# Autodesk Inventor assembly: Allocator for column chromatography
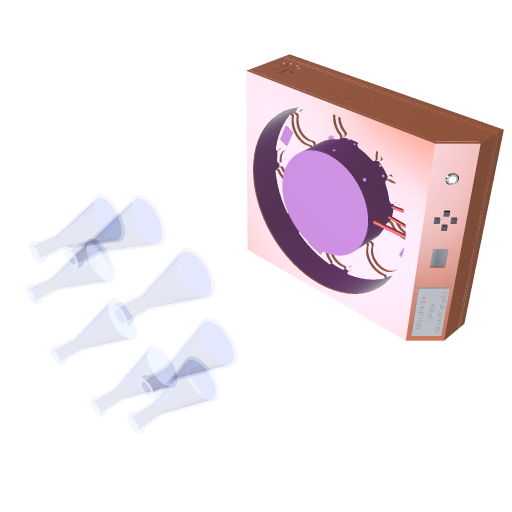
[picture p0: Inventor's stored thumbnail of the model, 512x512]
Saved by Autodesk Inventor 2023 (Build 270158000, 158)
## iProperties
Created: 2023-01-15
Part Number: Allocator for column chromatography
Document SubType Name: Assembly
Designer: Admin
Author: Admin
## Documents named in this file (38)
- C:\Users\aleks\OneDrive\Рабочий стол\Хроматографический сортировщик\Детали\Allocator for column chromatography.iam
- C:\Users\aleks\OneDrive\Рабочий стол\Хроматографический сортировщик\Детали\Барабан.ipt
- C:\Users\aleks\OneDrive\Рабочий стол\Хроматографический сортировщик\Детали\Корпус.ipt
- C:\Users\aleks\OneDrive\Рабочий стол\Хроматографический сортировщик\Детали\Покупные\Болт М5.ipt
- C:\Users\aleks\OneDrive\Рабочий стол\Хроматографический сортировщик\Детали\Покупные\Гайка М5 стопорная.ipt
- C:\Users\aleks\OneDrive\Рабочий стол\Хроматографический сортировщик\Детали\Покупные\Подшипник.ipt
- C:\Users\aleks\OneDrive\Рабочий стол\Хроматографический сортировщик\Детали\Короб подшипника.ipt
- C:\Users\aleks\OneDrive\Рабочий стол\Хроматографический сортировщик\Детали\Покупные\Гайка М3.ipt
- C:\Users\aleks\OneDrive\Рабочий стол\Хроматографический сортировщик\Детали\Покупные\Гайка М4.ipt
- C:\Users\aleks\OneDrive\Рабочий стол\Хроматографический сортировщик\Детали\Покупные\Гайка М6.ipt
- C:\Users\aleks\OneDrive\Рабочий стол\Хроматографический сортировщик\Детали\Покупные\Болт М6.ipt
- C:\Users\aleks\OneDrive\Рабочий стол\Хроматографический сортировщик\Детали\Крепёж оптического датчика.ipt
- C:\Users\aleks\OneDrive\Рабочий стол\Хроматографический сортировщик\Детали\Покупные\Болт М3.ipt
- C:\Users\aleks\OneDrive\Рабочий стол\Хроматографический сортировщик\Детали\Покупные\Болт М4.ipt
- C:\Users\aleks\OneDrive\Рабочий стол\Хроматографический сортировщик\Детали\Покупные\Шаговик\Вал.ipt
- C:\Users\aleks\OneDrive\Рабочий стол\Хроматографический сортировщик\Детали\Покупные\Шаговик\Шаговый мотор.ipt
- C:\Users\aleks\OneDrive\Рабочий стол\Хроматографический сортировщик\Детали\Покупные\Динамик\Динамик.ipt
- C:\Users\aleks\OneDrive\Рабочий стол\Хроматографический сортировщик\Детали\Покупные\Лазер маленький.ipt
- C:\Users\aleks\OneDrive\Рабочий стол\Хроматографический сортировщик\Детали\Покупные\Лазер.ipt
- C:\Users\aleks\OneDrive\Рабочий стол\Хроматографический сортировщик\Детали\Покупные\Оптический датчик.ipt
- C:\Users\aleks\OneDrive\Рабочий стол\Хроматографический сортировщик\Детали\Покупные\Свая.ipt
- C:\Users\aleks\OneDrive\Рабочий стол\Хроматографический сортировщик\Детали\Колесо энкодера.ipt
- C:\Users\aleks\OneDrive\Рабочий стол\Хроматографический сортировщик\Детали\Шевронная маленькая шестерня под мотор.ipt
- C:\Users\aleks\OneDrive\Рабочий стол\Хроматографический сортировщик\Детали\Шевронная планетарная шестерня.ipt
- C:\Users\aleks\OneDrive\Рабочий стол\Хроматографический сортировщик\Детали\Шевронная шестерня для энкодера.ipt
- C:\Users\aleks\OneDrive\Рабочий стол\Хроматографический сортировщик\Детали\Табличка.ipt
- C:\Users\aleks\OneDrive\Рабочий стол\Хроматографический сортировщик\Детали\Покупные\Дисплей.ipt
- C:\Users\aleks\OneDrive\Рабочий стол\Хроматографический сортировщик\Детали\Покупные\Кнопка.ipt
- C:\Users\aleks\OneDrive\Рабочий стол\Хроматографический сортировщик\Детали\Покупные\Кнопки на плате.iam
- C:\Users\aleks\OneDrive\Рабочий стол\Хроматографический сортировщик\Детали\Покупные\Плата главная.ipt
- C:\Users\aleks\OneDrive\Рабочий стол\Хроматографический сортировщик\Детали\Покупные\Разъём питания.ipt
- C:\Users\aleks\OneDrive\Рабочий стол\Хроматографический сортировщик\Детали\Покупные\Болт М2.ipt
- C:\Users\aleks\OneDrive\Рабочий стол\Хроматографический сортировщик\Детали\Покупные\Шаговик\Плата драйвера.ipt
- C:\Users\aleks\OneDrive\Рабочий стол\Хроматографический сортировщик\Детали\Покупные\Болт М3 4мм.ipt
- C:\Users\aleks\OneDrive\Рабочий стол\Хроматографический сортировщик\Детали\Колбы\Модель колба коническая 50мл.ipt
- C:\Users\aleks\OneDrive\Рабочий стол\Хроматографический сортировщик\Детали\Крышка анимации.ipt
- C:\Users\aleks\OneDrive\Рабочий стол\Хроматографический сортировщик\Детали\Покупные\Лазер 2.ipt
- C:\Users\aleks\OneDrive\Рабочий стол\Хроматографический сортировщик\Детали\Покупные\Лазер маленький 2.ipt
## Components (116 placed, 37 different names)
1. Корпус:1 — Совмещение:3, Заподлицо:6, Совмещение:36, Заподлицо:7, Совмещение:37, Угол:2, Заподлицо:8, Заподлицо:9, Совмещение:38, Угол:3, Совмещение:39, Заподлицо:10, Угол:4, Совмещение:40, Совмещение:41, Совмещение:42, Совмещение:43, Совмещение:44, Совмещение:45, Совмещение:46, Совмещение:47, Совмещение:48, Совмещение:49, Заподлицо:11, Заподлицо:12, Заподлицо:13, Заподлицо:14, Заподлицо:15, Заподлицо:16, Заподлицо:17, Заподлицо:18, Заподлицо:19, Заподлицо:20, Заподлицо:21, Заподлицо:22, Угол:5, Угол:6, Угол:7, Угол:8, Угол:9, Угол:10, Угол:11, Угол:12, Угол:13, Угол:14, Совмещение:50, Заподлицо:23, Угол:15, Совмещение:51, Совмещение:52, Совмещение:53, Совмещение:54, Заподлицо:24, Заподлицо:25, Заподлицо:26, Заподлицо:27, Угол:16, Угол:17, Угол:18, Угол:19, Совмещение:55, Совмещение:56, Заподлицо:28, Заподлицо:29, Угол:20, Угол:21, Совмещение:57, Совмещение:58, Заподлицо:30, Заподлицо:31, Угол:22, Угол:23, Совмещение:59, Совмещение:60, Совмещение:61, Совмещение:62, Совмещение:63, Совмещение:64, Совмещение:65, Совмещение:66, Заподлицо:32, Заподлицо:33, Заподлицо:34, Заподлицо:35, Заподлицо:36, Заподлицо:37, Заподлицо:38, Заподлицо:39, Совмещение:69, Совмещение:70, Совмещение:71, Совмещение:72, Совмещение:73, Совмещение:74, Совмещение:75, Совмещение:76, Совмещение:77, Совмещение:78, Совмещение:81, Совмещение:82, Совмещение:83, Совмещение:84, Совмещение:85, Совмещение:86, Угол:24, Угол:25, Заподлицо:40, Заподлицо:41, Совмещение:91, Совмещение:104, Совмещение:105, Совмещение:106, Совмещение:107, Совмещение:108, Совмещение:109, Совмещение:110, Совмещение:111, Совмещение:112, Совмещение:113, Совмещение:114, Совмещение:126, Совмещение:132, Совмещение:133, Совмещение:134, Совмещение:135, Угол:29, Совмещение:136, Совмещение:137, Совмещение:138, Совмещение:139, Совмещение:140, Совмещение:142, Совмещение:143, Совмещение:144, Совмещение:147, Совмещение:148, Совмещение:160, Совмещение:164, Совмещение:169, Совмещение:170, Совмещение:171, Совмещение:172, С поворотом:1, Угол:30, Совмещение:190, Заподлицо:67, Совмещение:191, Совмещение:192, Совмещение:193, Совмещение:194
2. Барабан:1 — Совмещение:3, Совмещение:4, Заподлицо:2, Совмещение:5, Совмещение:6, Совмещение:7, Заподлицо:3, Совмещение:8, Совмещение:9, Заподлицо:4, Совмещение:10, Совмещение:11, Заподлицо:5, Заподлицо:6, Совмещение:179, Совмещение:180, Совмещение:181, Совмещение:182, Совмещение:183, Совмещение:184, Совмещение:185, Совмещение:186, Совмещение:187, Касательность:1, Касательность:2, ЗубчПер:5, С поворотом:1, Угол:30, Совмещение:188, Совмещение:189, ЗубчПер:6
3. Болт М5:1 — Совмещение:19, Совмещение:28
4. Гайка М5 стопорная:1 — Совмещение:23, Совмещение:31
5. Подшипник:1 — Совмещение:15, Совмещение:19, Совмещение:22, Совмещение:25
6. Болт М5:2 — Совмещение:16, Совмещение:20, Совмещение:32
7. Гайка М5 стопорная:2 — Совмещение:20, Совмещение:33
8. Подшипник:2 — Совмещение:12, Совмещение:16, Совмещение:27
9. Болт М5:3 — Совмещение:17, Совмещение:21, Совмещение:34
10. Гайка М5 стопорная:3 — Совмещение:21, Совмещение:35
11. Подшипник:3 — Совмещение:13, Совмещение:17, Совмещение:24
12. Болт М5:4 — Совмещение:18, Совмещение:23, Совмещение:30
13. Гайка М5 стопорная:4 — Совмещение:22, Совмещение:29
14. Подшипник:4 — Совмещение:14, Совмещение:18, Совмещение:26
15. Короб подшипника:1 — Совмещение:8, Совмещение:9, Заподлицо:4, Совмещение:12, Совмещение:27, Совмещение:32, Совмещение:33
16. Короб подшипника:2 — Совмещение:6, Совмещение:7, Заподлицо:3, Совмещение:13, Совмещение:24, Совмещение:34, Совмещение:35
17. Короб подшипника:3 — Совмещение:4, Заподлицо:2, Совмещение:5, Совмещение:15, Совмещение:25, Совмещение:28, Совмещение:29
18. Короб подшипника:4 — Совмещение:10, Совмещение:11, Заподлицо:5, Совмещение:14, Совмещение:26, Совмещение:30, Совмещение:31
19. Подшипник:5 — Совмещение:36, Заподлицо:7, Совмещение:119
20. Гайка М3:1 — Совмещение:41, Заподлицо:13, Угол:6
21. Гайка М3:2 — Совмещение:50, Заподлицо:23, Угол:15
22. Гайка М3:3 — Совмещение:40, Заподлицо:14, Угол:5
23. Гайка М3:4 — Совмещение:43, Заподлицо:22, Угол:8
24. Гайка М3:5 — Совмещение:47, Заподлицо:16, Угол:11
25. Гайка М3:6 — Совмещение:48, Заподлицо:17, Угол:13
26. Гайка М3:7 — Совмещение:37, Угол:2, Заподлицо:8
27. Гайка М3:8 — Заподлицо:9, Совмещение:38, Угол:3, Заподлицо:12
28. Гайка М3:9 — Совмещение:44, Заподлицо:19, Угол:9
29. Гайка М3:11 — Совмещение:49, Заподлицо:18, Угол:14
30. Гайка М3:12 — Совмещение:39, Заподлицо:10, Угол:4, Заподлицо:11
31. Гайка М3:13 — Совмещение:42, Заподлицо:21, Угол:7
32. Гайка М3:14 — Совмещение:45, Заподлицо:20, Угол:10
33. Гайка М3:15 — Совмещение:46, Заподлицо:15, Угол:12
34. Гайка М4:1 — Совмещение:56, Заподлицо:28, Угол:21
35. Гайка М6:1 — Совмещение:53, Заподлицо:26, Угол:17
36. Гайка М4:2 — Совмещение:55, Заподлицо:29, Угол:20
37. Гайка М6:2 — Совмещение:52, Заподлицо:24, Угол:19
38. Гайка М6:3 — Совмещение:51, Заподлицо:25, Угол:18
39. Гайка М6:4 — Совмещение:54, Заподлицо:27, Угол:16
40. Болт М6:1 — Совмещение:61, Заподлицо:34
41. Болт М6:2 — Совмещение:60, Заподлицо:39
42. Гайка М6:5 — Совмещение:57, Заподлицо:31, Угол:22
43. Гайка М6:6 — Совмещение:58, Заподлицо:30, Угол:23
44. Болт М6:3 — Совмещение:62, Заподлицо:37
45. Болт М6:4 — Совмещение:59, Заподлицо:38
46. Болт М6:5 — Совмещение:65, Заподлицо:33
47. Болт М6:6 — Совмещение:64, Заподлицо:35, Совмещение:90
48. Болт М6:7 — Совмещение:66, Заподлицо:32
49. Болт М6:8 — Совмещение:63, Заподлицо:36, Совмещение:89
50. Крепёж оптического датчика:1 — Совмещение:69, Совмещение:87, Совмещение:88, Совмещение:115, Совмещение:116, Совмещение:120, Совмещение:122, Совмещение:123, Угол:26, Угол:27, Совмещение:167, Совмещение:168
51. Болт М3:1 — Совмещение:81, Совмещение:84
52. Болт М3:2 — Совмещение:87, Совмещение:167, Совмещение:171
53. Болт М3:3 — Совмещение:72, Заподлицо:53, Заподлицо:54, Совмещение:152, Совмещение:157
54. Болт М3:4 — Совмещение:78, Заподлицо:43
55. Болт М3:5 — Совмещение:82, Совмещение:83
56. Болт М3:6 — Совмещение:73, Заподлицо:53, Совмещение:153, Совмещение:158
57. Болт М3:7 — Совмещение:76, Заподлицо:44, Заподлицо:45, Совмещение:161
58. Болт М3:8 — Совмещение:70, Совмещение:86
59. Болт М3:9 — Совмещение:75, Заподлицо:52, Заподлицо:54, Совмещение:155
60. Болт М3:10 — Совмещение:74, Заподлицо:52, Совмещение:154, Совмещение:156
61. Болт М3:11 — Совмещение:77, Заподлицо:43, Заподлицо:44, Совмещение:162, Совмещение:163
62. Болт М3:12 — Совмещение:88, Совмещение:168, Совмещение:172
63. Болт М3:13 — Совмещение:71, Совмещение:85
64. Гайка М6:7 — Совмещение:90, Угол:24, Заподлицо:41
65. Гайка М6:8 — Совмещение:89, Угол:25, Заподлицо:40
66. Болт М3:14 — Совмещение:91, Заподлицо:45
67. Болт М4:1 — Совмещение:100, Совмещение:102, Совмещение:169
68. Болт М4:2 — Совмещение:101, Совмещение:103, Совмещение:170
69. Вал:1 — Совмещение:98, Совмещение:99, Совмещение:130, Угол:28, Совмещение:131
70. Шаговый мотор:1 — Совмещение:98, Совмещение:99, Совмещение:100, Совмещение:101, Совмещение:102, Совмещение:103, Совмещение:104
71. Динамик:1 — Совмещение:106, Совмещение:108
72. Динамик:2 — Совмещение:105, Совмещение:107
73. Лазер маленький:1 — Совмещение:111, Совмещение:112
74. Лазер маленький:2 — Совмещение:110, Совмещение:113, Касательность:1, Касательность:2
75. Лазер:1 — Совмещение:109, Совмещение:114
76. Оптический датчик:1 — Совмещение:120, Совмещение:121, Совмещение:122, Совмещение:124, Совмещение:125, Совмещение:129
77. Свая:1 — Совмещение:119, Совмещение:126, Совмещение:127, Совмещение:128, ЗубчПер:1
78. Болт М3:15 — Совмещение:116, Совмещение:118, Совмещение:121, Совмещение:125
79. Гайка М3:16 — Совмещение:118, Заподлицо:46, Угол:27
80. Болт М3:16 — Совмещение:115, Совмещение:117, Совмещение:124
81. Гайка М3:17 — Совмещение:117, Заподлицо:46, Совмещение:123, Угол:26
82. Колесо энкодера:1 — Совмещение:127, Совмещение:129, ЗубчПер:3, Совмещение:173, Совмещение:174
83. Шевронная маленькая шестерня под мотор:1 — Совмещение:130, Угол:28, Совмещение:131, Заподлицо:47, Заподлицо:48, ЗубчПер:2, ЗубчПер:4
84. Шевронная шестерня для энкодера:1 — Совмещение:128, Заподлицо:47, ЗубчПер:1, ЗубчПер:2, ЗубчПер:3, Совмещение:175, Совмещение:176
85. Шевронная планетарная шестерня:1 — Совмещение:132, Заподлицо:48, ЗубчПер:4, ЗубчПер:5
86. Табличка:1 — Совмещение:135, Угол:29, Совмещение:136, Совмещение:137
87. Кнопка:1 — Совмещение:138, Совмещение:139
88. Кнопки на плате:1 [sub-assembly] — Совмещение:140, Совмещение:142, Совмещение:143
89. Плата главная:1 — Совмещение:152, Совмещение:153, Совмещение:154, Совмещение:159
90. Разъём питания:1 — Совмещение:133, Совмещение:134
91. Болт М2:1 — Заподлицо:49, Заподлицо:50, Заподлицо:51, Совмещение:145, Совмещение:147, Совмещение:151
92. Болт М2:2 — Заподлицо:49, Совмещение:149
93. Болт М2:3 — Заподлицо:51, Совмещение:146, Совмещение:148
94. Болт М2:4 — Заподлицо:50, Совмещение:150
95. Дисплей:1 — Совмещение:144, Совмещение:145, Совмещение:146, Совмещение:149, Совмещение:150, Совмещение:151
96. Гайка М3:18 — Совмещение:155, Заподлицо:56, Заподлицо:57
97. Гайка М3:19 — Совмещение:156, Заподлицо:55, Заподлицо:57
98. Гайка М3:20 — Совмещение:157, Заподлицо:56
99. Гайка М3:21 — Совмещение:158, Заподлицо:55, Совмещение:159, Совмещение:160
100. Плата драйвера:1 — Совмещение:161, Совмещение:162, Совмещение:163, Совмещение:164
101. Болт М3 4мм:1 — Совмещение:173, Совмещение:174
102. Болт М3 4мм:2 — Совмещение:175, Совмещение:176
103. Подшипник:6
104. Подшипник:7
105. Модель колба коническая 50мл:2 — Совмещение:180, Заподлицо:61, Заподлицо:62
106. Модель колба коническая 50мл:3 — Совмещение:181, Заподлицо:66
107. Модель колба коническая 50мл:4 — Совмещение:182, Заподлицо:60, Заподлицо:61
108. Модель колба коническая 50мл:5 — Совмещение:186, Заподлицо:64
109. Модель колба коническая 50мл:6 — Совмещение:183, Заподлицо:60
110. Модель колба коническая 50мл:7 — Совмещение:184, Заподлицо:65
111. Модель колба коническая 50мл:8 — Совмещение:185, Заподлицо:63
112. Модель колба коническая 50мл:9 — Совмещение:179, Заподлицо:62, Заподлицо:63, Заподлицо:64, Заподлицо:65, Заподлицо:66, Совмещение:187
113. Крышка анимации:1 — Совмещение:188, Совмещение:189, ЗубчПер:6
114. Лазер 2:1 — Совмещение:190, Заподлицо:67
115. Лазер маленький 2:1 — Совмещение:191, Совмещение:194
116. Лазер маленький 2:2 — Совмещение:192, Совмещение:193
## Relationships (278: Mate 177, Flush 63, Angle 29, RelateRotation 6, Tangent 2, RevoluteJoint 1)
- Совмещение:3 [Mate]: Корпус:1 ↔ Барабан:1
- Совмещение:4 [Mate] (0.1 mm): Барабан:1 ↔ Короб подшипника:3
- Заподлицо:2 [Flush]: Барабан:1 ↔ Короб подшипника:3
- Совмещение:5 [Mate] (0.1 mm): Барабан:1 ↔ Короб подшипника:3
- Совмещение:6 [Mate] (0.1 mm): Барабан:1 ↔ Короб подшипника:2
- Совмещение:7 [Mate] (0.1 mm): Барабан:1 ↔ Короб подшипника:2
- Заподлицо:3 [Flush]: Барабан:1 ↔ Короб подшипника:2
- Совмещение:8 [Mate] (0.1 mm): Барабан:1 ↔ Короб подшипника:1
- Совмещение:9 [Mate] (0.1 mm): Барабан:1 ↔ Короб подшипника:1
- Заподлицо:4 [Flush]: Барабан:1 ↔ Короб подшипника:1
- Совмещение:10 [Mate] (0.1 mm): Барабан:1 ↔ Короб подшипника:4
- Совмещение:11 [Mate] (0.1 mm): Барабан:1 ↔ Короб подшипника:4
- Заподлицо:5 [Flush]: Барабан:1 ↔ Короб подшипника:4
- Совмещение:12 [Mate]: Подшипник:2 ↔ Короб подшипника:1
- Совмещение:13 [Mate]: Подшипник:3 ↔ Короб подшипника:2
- Совмещение:14 [Mate]: Подшипник:4 ↔ Короб подшипника:4
- Совмещение:15 [Mate]: Подшипник:1 ↔ Короб подшипника:3
- Совмещение:16 [Mate]: Болт М5:2 ↔ Подшипник:2
- Совмещение:17 [Mate]: Болт М5:3 ↔ Подшипник:3
- Совмещение:18 [Mate]: Болт М5:4 ↔ Подшипник:4
- Совмещение:19 [Mate]: Болт М5:1 ↔ Подшипник:1
- Совмещение:20 [Mate]: Болт М5:2 ↔ Гайка М5 стопорная:2
- Совмещение:21 [Mate]: Болт М5:3 ↔ Гайка М5 стопорная:3
- Совмещение:22 [Mate]: Подшипник:1 ↔ Гайка М5 стопорная:4
- Совмещение:23 [Mate]: Гайка М5 стопорная:1 ↔ Болт М5:4
- Совмещение:24 [Mate] (0.5 mm): Подшипник:3 ↔ Короб подшипника:2
- Совмещение:25 [Mate] (0.5 mm): Подшипник:1 ↔ Короб подшипника:3
- Совмещение:26 [Mate] (0.5 mm): Подшипник:4 ↔ Короб подшипника:4
- Совмещение:27 [Mate] (0.5 mm): Подшипник:2 ↔ Короб подшипника:1
- Совмещение:28 [Mate]: Болт М5:1 ↔ Короб подшипника:3
- Совмещение:29 [Mate]: Гайка М5 стопорная:4 ↔ Короб подшипника:3
- Совмещение:30 [Mate]: Болт М5:4 ↔ Короб подшипника:4
- Совмещение:31 [Mate]: Гайка М5 стопорная:1 ↔ Короб подшипника:4
- Совмещение:32 [Mate]: Болт М5:2 ↔ Короб подшипника:1
- Совмещение:33 [Mate]: Гайка М5 стопорная:2 ↔ Короб подшипника:1
- Совмещение:34 [Mate]: Болт М5:3 ↔ Короб подшипника:2
- Совмещение:35 [Mate]: Гайка М5 стопорная:3 ↔ Короб подшипника:2
- Заподлицо:6 [Flush]: Корпус:1 ↔ Барабан:1
- Совмещение:36 [Mate]: Корпус:1 ↔ Подшипник:5
- Заподлицо:7 [Flush]: Корпус:1 ↔ Подшипник:5
- Совмещение:37 [Mate]: Корпус:1 ↔ Гайка М3:7
- Угол:2 [Angle] (0 deg): Корпус:1 ↔ Гайка М3:7
- Заподлицо:8 [Flush]: Корпус:1 ↔ Гайка М3:7
- Заподлицо:9 [Flush]: Корпус:1 ↔ Гайка М3:8
- Совмещение:38 [Mate]: Корпус:1 ↔ Гайка М3:8
- Угол:3 [Angle] (0 deg): Корпус:1 ↔ Гайка М3:8
- Совмещение:39 [Mate]: Корпус:1 ↔ Гайка М3:12
- Заподлицо:10 [Flush]: Корпус:1 ↔ Гайка М3:12
- Угол:4 [Angle] (0 deg): Корпус:1 ↔ Гайка М3:12
- Совмещение:40 [Mate]: Корпус:1 ↔ Гайка М3:3
- Совмещение:41 [Mate]: Корпус:1 ↔ Гайка М3:1
- Совмещение:42 [Mate]: Корпус:1 ↔ Гайка М3:13
- Совмещение:43 [Mate]: Корпус:1 ↔ Гайка М3:4
- Совмещение:44 [Mate]: Корпус:1 ↔ Гайка М3:9
- Совмещение:45 [Mate]: Корпус:1 ↔ Гайка М3:14
- Совмещение:46 [Mate]: Корпус:1 ↔ Гайка М3:15
- Совмещение:47 [Mate]: Корпус:1 ↔ Гайка М3:5
- Совмещение:48 [Mate]: Корпус:1 ↔ Гайка М3:6
- Совмещение:49 [Mate]: Корпус:1 ↔ Гайка М3:11
- Заподлицо:11 [Flush]: Корпус:1 ↔ Гайка М3:12
- Заподлицо:12 [Flush]: Корпус:1 ↔ Гайка М3:8
- Заподлицо:13 [Flush]: Корпус:1 ↔ Гайка М3:1
- Заподлицо:14 [Flush]: Корпус:1 ↔ Гайка М3:3
- Заподлицо:15 [Flush]: Корпус:1 ↔ Гайка М3:15
- Заподлицо:16 [Flush]: Корпус:1 ↔ Гайка М3:5
- Заподлицо:17 [Flush]: Корпус:1 ↔ Гайка М3:6
- Заподлицо:18 [Flush]: Корпус:1 ↔ Гайка М3:11
- Заподлицо:19 [Flush]: Корпус:1 ↔ Гайка М3:9
- Заподлицо:20 [Flush]: Корпус:1 ↔ Гайка М3:14
- Заподлицо:21 [Flush]: Корпус:1 ↔ Гайка М3:13
- Заподлицо:22 [Flush]: Корпус:1 ↔ Гайка М3:4
- Угол:5 [Angle] (0 deg): Корпус:1 ↔ Гайка М3:3
- Угол:6 [Angle] (0 deg): Корпус:1 ↔ Гайка М3:1
- Угол:7 [Angle] (0 deg): Корпус:1 ↔ Гайка М3:13
- Угол:8 [Angle] (0 deg): Корпус:1 ↔ Гайка М3:4
- Угол:9 [Angle] (0 deg): Корпус:1 ↔ Гайка М3:9
- Угол:10 [Angle] (0 deg): Корпус:1 ↔ Гайка М3:14
- Угол:11 [Angle] (0 deg): Корпус:1 ↔ Гайка М3:5
- Угол:12 [Angle] (0 deg): Корпус:1 ↔ Гайка М3:15
- Угол:13 [Angle] (0 deg): Корпус:1 ↔ Гайка М3:6
- Угол:14 [Angle] (0 deg): Корпус:1 ↔ Гайка М3:11
- Совмещение:50 [Mate]: Корпус:1 ↔ Гайка М3:2
- Заподлицо:23 [Flush]: Корпус:1 ↔ Гайка М3:2
- Угол:15 [Angle] (0 deg): Корпус:1 ↔ Гайка М3:2
- Совмещение:51 [Mate]: Корпус:1 ↔ Гайка М6:3
- Совмещение:52 [Mate]: Корпус:1 ↔ Гайка М6:2
- Совмещение:53 [Mate]: Корпус:1 ↔ Гайка М6:1
- Совмещение:54 [Mate]: Корпус:1 ↔ Гайка М6:4
- Заподлицо:24 [Flush]: Корпус:1 ↔ Гайка М6:2
- Заподлицо:25 [Flush]: Корпус:1 ↔ Гайка М6:3
- Заподлицо:26 [Flush]: Корпус:1 ↔ Гайка М6:1
- Заподлицо:27 [Flush]: Корпус:1 ↔ Гайка М6:4
- Угол:16 [Angle] (0 deg): Корпус:1 ↔ Гайка М6:4
- Угол:17 [Angle] (0 deg): Корпус:1 ↔ Гайка М6:1
- Угол:18 [Angle] (0 deg): Корпус:1 ↔ Гайка М6:3
- Угол:19 [Angle] (0 deg): Корпус:1 ↔ Гайка М6:2
- Совмещение:55 [Mate]: Корпус:1 ↔ Гайка М4:2
- Совмещение:56 [Mate]: Корпус:1 ↔ Гайка М4:1
- Заподлицо:28 [Flush]: Корпус:1 ↔ Гайка М4:1
- Заподлицо:29 [Flush]: Корпус:1 ↔ Гайка М4:2
- Угол:20 [Angle] (0 deg): Корпус:1 ↔ Гайка М4:2
- Угол:21 [Angle] (0 deg): Корпус:1 ↔ Гайка М4:1
- Совмещение:57 [Mate]: Корпус:1 ↔ Гайка М6:5
- Совмещение:58 [Mate]: Корпус:1 ↔ Гайка М6:6
- Заподлицо:30 [Flush]: Корпус:1 ↔ Гайка М6:6
- Заподлицо:31 [Flush]: Корпус:1 ↔ Гайка М6:5
- Угол:22 [Angle] (0 deg): Корпус:1 ↔ Гайка М6:5
- Угол:23 [Angle] (0 deg): Корпус:1 ↔ Гайка М6:6
- Совмещение:59 [Mate]: Корпус:1 ↔ Болт М6:4
- Совмещение:60 [Mate]: Корпус:1 ↔ Болт М6:2
- Совмещение:61 [Mate]: Корпус:1 ↔ Болт М6:1
- Совмещение:62 [Mate]: Корпус:1 ↔ Болт М6:3
- Совмещение:63 [Mate]: Корпус:1 ↔ Болт М6:8
- Совмещение:64 [Mate]: Корпус:1 ↔ Болт М6:6
- Совмещение:65 [Mate]: Корпус:1 ↔ Болт М6:5
- Совмещение:66 [Mate]: Корпус:1 ↔ Болт М6:7
- Заподлицо:32 [Flush]: Корпус:1 ↔ Болт М6:7
- Заподлицо:33 [Flush]: Корпус:1 ↔ Болт М6:5
- Заподлицо:34 [Flush]: Корпус:1 ↔ Болт М6:1
- Заподлицо:35 [Flush]: Корпус:1 ↔ Болт М6:6
- Заподлицо:36 [Flush]: Корпус:1 ↔ Болт М6:8
- Заподлицо:37 [Flush]: Корпус:1 ↔ Болт М6:3
- Заподлицо:38 [Flush]: Корпус:1 ↔ Болт М6:4
- Заподлицо:39 [Flush]: Корпус:1 ↔ Болт М6:2
- Совмещение:69 [Mate]: Корпус:1 ↔ Крепёж оптического датчика:1
- Совмещение:70 [Mate]: Корпус:1 ↔ Болт М3:8
- Совмещение:71 [Mate]: Корпус:1 ↔ Болт М3:13
- Совмещение:72 [Mate]: Корпус:1 ↔ Болт М3:3
- Совмещение:73 [Mate]: Корпус:1 ↔ Болт М3:6
- Совмещение:74 [Mate]: Корпус:1 ↔ Болт М3:10
- Совмещение:75 [Mate]: Корпус:1 ↔ Болт М3:9
- Совмещение:76 [Mate]: Корпус:1 ↔ Болт М3:7
- Совмещение:77 [Mate]: Корпус:1 ↔ Болт М3:11
- Совмещение:78 [Mate]: Корпус:1 ↔ Болт М3:4
- Совмещение:81 [Mate]: Корпус:1 ↔ Болт М3:1
- Совмещение:82 [Mate]: Корпус:1 ↔ Болт М3:5
- Совмещение:83 [Mate]: Корпус:1 ↔ Болт М3:5
- Совмещение:84 [Mate]: Корпус:1 ↔ Болт М3:1
- Совмещение:85 [Mate]: Корпус:1 ↔ Болт М3:13
- Совмещение:86 [Mate]: Корпус:1 ↔ Болт М3:8
- Совмещение:87 [Mate]: Крепёж оптического датчика:1 ↔ Болт М3:2
- Совмещение:88 [Mate]: Крепёж оптического датчика:1 ↔ Болт М3:12
- Совмещение:89 [Mate]: Болт М6:8 ↔ Гайка М6:8
- Совмещение:90 [Mate]: Болт М6:6 ↔ Гайка М6:7
- Угол:24 [Angle] (0 deg): Корпус:1 ↔ Гайка М6:7
- Угол:25 [Angle] (0 deg): Корпус:1 ↔ Гайка М6:8
- Заподлицо:40 [Flush]: Корпус:1 ↔ Гайка М6:8
- Заподлицо:41 [Flush]: Корпус:1 ↔ Гайка М6:7
- Совмещение:91 [Mate]: Корпус:1 ↔ Болт М3:14
- Заподлицо:43 [Flush]: Болт М3:4 ↔ Болт М3:11
- Заподлицо:44 [Flush]: Болт М3:7 ↔ Болт М3:11
- Заподлицо:45 [Flush]: Болт М3:7 ↔ Болт М3:14
- Совмещение:98 [Mate]: Вал:1 ↔ Шаговый мотор:1
- Совмещение:99 [Mate]: Вал:1 ↔ Шаговый мотор:1
- Совмещение:100 [Mate]: Болт М4:1 ↔ Шаговый мотор:1
- Совмещение:101 [Mate]: Болт М4:2 ↔ Шаговый мотор:1
- Совмещение:102 [Mate]: Болт М4:1 ↔ Шаговый мотор:1
- Совмещение:103 [Mate]: Болт М4:2 ↔ Шаговый мотор:1
- Совмещение:104 [Mate]: Корпус:1 ↔ Шаговый мотор:1
- Совмещение:105 [Mate]: Корпус:1 ↔ Динамик:2
- Совмещение:106 [Mate]: Корпус:1 ↔ Динамик:1
- Совмещение:107 [Mate]: Корпус:1 ↔ Динамик:2
- Совмещение:108 [Mate]: Корпус:1 ↔ Динамик:1
- Совмещение:109 [Mate]: Корпус:1 ↔ Лазер:1
- Совмещение:110 [Mate]: Корпус:1 ↔ Лазер маленький:2
- Совмещение:111 [Mate]: Корпус:1 ↔ Лазер маленький:1
- Совмещение:112 [Mate]: Корпус:1 ↔ Лазер маленький:1
- Совмещение:113 [Mate]: Корпус:1 ↔ Лазер маленький:2
- Совмещение:114 [Mate]: Корпус:1 ↔ Лазер:1
- Совмещение:115 [Mate]: Крепёж оптического датчика:1 ↔ Болт М3:16
- Совмещение:116 [Mate]: Крепёж оптического датчика:1 ↔ Болт М3:15
- Совмещение:117 [Mate]: Болт М3:16 ↔ Гайка М3:17
- Совмещение:118 [Mate]: Болт М3:15 ↔ Гайка М3:16
- Совмещение:119 [Mate]: Подшипник:5 ↔ Свая:1
- Совмещение:120 [Mate]: Крепёж оптического датчика:1 ↔ Оптический датчик:1
- Совмещение:121 [Mate]: Оптический датчик:1 ↔ Болт М3:15
- Совмещение:122 [Mate]: Крепёж оптического датчика:1 ↔ Оптический датчик:1
- Заподлицо:46 [Flush]: Гайка М3:16 ↔ Гайка М3:17
- Совмещение:123 [Mate]: Крепёж оптического датчика:1 ↔ Гайка М3:17
- Угол:26 [Angle] (0 deg): Крепёж оптического датчика:1 ↔ Гайка М3:17
- Угол:27 [Angle] (0 deg): Крепёж оптического датчика:1 ↔ Гайка М3:16
- Совмещение:124 [Mate]: Оптический датчик:1 ↔ Болт М3:16
- Совмещение:125 [Mate]: Оптический датчик:1 ↔ Болт М3:15
- Совмещение:126 [Mate]: Корпус:1 ↔ Свая:1
- Совмещение:127 [Mate]: Свая:1 ↔ Колесо энкодера:1
- Совмещение:128 [Mate]: Свая:1 ↔ Шевронная шестерня для энкодера:1
- Совмещение:129 [Mate] (2 mm): Оптический датчик:1 ↔ Колесо энкодера:1
- Совмещение:130 [Mate]: Вал:1 ↔ Шевронная маленькая шестерня под мотор:1
- Угол:28 [Angle] (0 deg): Вал:1 ↔ Шевронная маленькая шестерня под мотор:1
- Совмещение:131 [Mate]: Вал:1 ↔ Шевронная маленькая шестерня под мотор:1
- Заподлицо:47 [Flush]: Шевронная маленькая шестерня под мотор:1 ↔ Шевронная шестерня для энкодера:1
- Совмещение:132 [Mate]: Корпус:1 ↔ Шевронная планетарная шестерня:1
- Заподлицо:48 [Flush]: Шевронная маленькая шестерня под мотор:1 ↔ Шевронная планетарная шестерня:1
- ЗубчПер:1 [RelateRotation] (1 ul): Свая:1 ↔ Шевронная шестерня для энкодера:1
- ЗубчПер:2 [RelateRotation] (1 ul): Шевронная маленькая шестерня под мотор:1 ↔ Шевронная шестерня для энкодера:1
- ЗубчПер:3 [RelateRotation] (1 ul): Колесо энкодера:1 ↔ Шевронная шестерня для энкодера:1
- ЗубчПер:4 [RelateRotation] (0.375 ul): Шевронная маленькая шестерня под мотор:1 ↔ Шевронная планетарная шестерня:1
- Совмещение:133 [Mate]: Корпус:1 ↔ Разъём питания:1
- Совмещение:134 [Mate]: Корпус:1 ↔ Разъём питания:1
- Совмещение:135 [Mate]: Корпус:1 ↔ Табличка:1
- Угол:29 [Angle] (0 deg): Корпус:1 ↔ Табличка:1
- Совмещение:136 [Mate] (5.127 mm): Корпус:1 ↔ Табличка:1
- Совмещение:137 [Mate] (10 mm): Корпус:1 ↔ Табличка:1
- Совмещение:138 [Mate]: Корпус:1 ↔ Кнопка:1
- Совмещение:139 [Mate]: Корпус:1 ↔ Кнопка:1
- Совмещение:140 [Mate]: Корпус:1 ↔ Кнопки на плате:1
- Совмещение:142 [Mate] (0.05 mm): Корпус:1 ↔ Кнопки на плате:1
- Совмещение:143 [Mate] (0.05 mm): Корпус:1 ↔ Кнопки на плате:1
- Заподлицо:49 [Flush]: Болт М2:1 ↔ Болт М2:2
- Заподлицо:50 [Flush]: Болт М2:1 ↔ Болт М2:4
- Заподлицо:51 [Flush]: Болт М2:1 ↔ Болт М2:3
- Совмещение:144 [Mate]: Корпус:1 ↔ Дисплей:1
- Совмещение:145 [Mate]: Болт М2:1 ↔ Дисплей:1
- Совмещение:146 [Mate]: Болт М2:3 ↔ Дисплей:1
- Совмещение:147 [Mate]: Корпус:1 ↔ Болт М2:1
- Совмещение:148 [Mate]: Корпус:1 ↔ Болт М2:3
- Совмещение:149 [Mate]: Болт М2:2 ↔ Дисплей:1
- Совмещение:150 [Mate]: Болт М2:4 ↔ Дисплей:1
- Совмещение:151 [Mate]: Болт М2:1 ↔ Дисплей:1
- Заподлицо:52 [Flush]: Болт М3:9 ↔ Болт М3:10
- Заподлицо:53 [Flush]: Болт М3:3 ↔ Болт М3:6
- Заподлицо:54 [Flush]: Болт М3:3 ↔ Болт М3:9
- Совмещение:152 [Mate]: Болт М3:3 ↔ Плата главная:1
- Совмещение:153 [Mate]: Болт М3:6 ↔ Плата главная:1
- Совмещение:154 [Mate]: Болт М3:10 ↔ Плата главная:1
- Совмещение:155 [Mate]: Болт М3:9 ↔ Гайка М3:18
- Совмещение:156 [Mate]: Болт М3:10 ↔ Гайка М3:19
- Совмещение:157 [Mate]: Болт М3:3 ↔ Гайка М3:20
- Совмещение:158 [Mate]: Болт М3:6 ↔ Гайка М3:21
- Заподлицо:55 [Flush]: Гайка М3:19 ↔ Гайка М3:21
- Заподлицо:56 [Flush]: Гайка М3:18 ↔ Гайка М3:20
- Заподлицо:57 [Flush]: Гайка М3:18 ↔ Гайка М3:19
- Совмещение:159 [Mate]: Плата главная:1 ↔ Гайка М3:21
- Совмещение:160 [Mate]: Корпус:1 ↔ Гайка М3:21
- Совмещение:161 [Mate]: Болт М3:7 ↔ Плата драйвера:1
- Совмещение:162 [Mate]: Болт М3:11 ↔ Плата драйвера:1
- Совмещение:163 [Mate]: Болт М3:11 ↔ Плата драйвера:1
- Совмещение:164 [Mate]: Корпус:1 ↔ Плата драйвера:1
- Совмещение:167 [Mate]: Крепёж оптического датчика:1 ↔ Болт М3:2
- Совмещение:168 [Mate]: Крепёж оптического датчика:1 ↔ Болт М3:12
- Совмещение:169 [Mate]: Корпус:1 ↔ Болт М4:1
- Совмещение:170 [Mate]: Корпус:1 ↔ Болт М4:2
- Совмещение:171 [Mate]: Корпус:1 ↔ Болт М3:2
- Совмещение:172 [Mate]: Корпус:1 ↔ Болт М3:12
- Совмещение:173 [Mate]: Колесо энкодера:1 ↔ Болт М3 4мм:1
- Совмещение:174 [Mate] (2.5 mm): Колесо энкодера:1 ↔ Болт М3 4мм:1
- Совмещение:175 [Mate]: Шевронная шестерня для энкодера:1 ↔ Болт М3 4мм:2
- Совмещение:176 [Mate] (2.5 mm): Шевронная шестерня для энкодера:1 ↔ Болт М3 4мм:2
- Совмещение:179 [Mate]: Барабан:1 ↔ Модель колба коническая 50мл:9
- Совмещение:180 [Mate]: Барабан:1 ↔ Модель колба коническая 50мл:2
- Совмещение:181 [Mate]: Барабан:1 ↔ Модель колба коническая 50мл:3
- Совмещение:182 [Mate]: Барабан:1 ↔ Модель колба коническая 50мл:4
- Совмещение:183 [Mate]: Барабан:1 ↔ Модель колба коническая 50мл:6
- Совмещение:184 [Mate]: Барабан:1 ↔ Модель колба коническая 50мл:7
- Совмещение:185 [Mate]: Барабан:1 ↔ Модель колба коническая 50мл:8
- Совмещение:186 [Mate]: Барабан:1 ↔ Модель колба коническая 50мл:5
- Заподлицо:60 [Flush]: Модель колба коническая 50мл:4 ↔ Модель колба коническая 50мл:6
- Заподлицо:61 [Flush]: Модель колба коническая 50мл:2 ↔ Модель колба коническая 50мл:4
- Заподлицо:62 [Flush]: Модель колба коническая 50мл:2 ↔ Модель колба коническая 50мл:9
- Заподлицо:63 [Flush]: Модель колба коническая 50мл:8 ↔ Модель колба коническая 50мл:9
- Заподлицо:64 [Flush]: Модель колба коническая 50мл:5 ↔ Модель колба коническая 50мл:9
- Заподлицо:65 [Flush]: Модель колба коническая 50мл:7 ↔ Модель колба коническая 50мл:9
- Заподлицо:66 [Flush]: Модель колба коническая 50мл:3 ↔ Модель колба коническая 50мл:9
- Совмещение:187 [Mate] (300 mm): Барабан:1 ↔ Модель колба коническая 50мл:9
- Касательность:1 [Tangent]: Барабан:1 ↔ Лазер маленький:2
- Касательность:2 [Tangent]: Барабан:1 ↔ Лазер маленький:2
- ЗубчПер:5 [RelateRotation] (1 ul): Барабан:1 ↔ Шевронная планетарная шестерня:1
- С поворотом:1 [RevoluteJoint]: Корпус:1 ↔ Барабан:1
- Угол:30 [Angle] (0 deg): Корпус:1 ↔ Барабан:1
- Совмещение:188 [Mate]: Барабан:1 ↔ Крышка анимации:1
- Совмещение:189 [Mate]: Барабан:1 ↔ Крышка анимации:1
- ЗубчПер:6 [RelateRotation] (1 ul): Барабан:1 ↔ Крышка анимации:1
- Совмещение:190 [Mate]: Корпус:1 ↔ Лазер 2:1
- Заподлицо:67 [Flush]: Корпус:1 ↔ Лазер 2:1
- Совмещение:191 [Mate]: Корпус:1 ↔ Лазер маленький 2:1
- Совмещение:192 [Mate]: Корпус:1 ↔ Лазер маленький 2:2
- Совмещение:193 [Mate]: Корпус:1 ↔ Лазер маленький 2:2
- Совмещение:194 [Mate]: Корпус:1 ↔ Лазер маленький 2:1
